# Autodesk Inventor assembly: Elevator Car with Plate
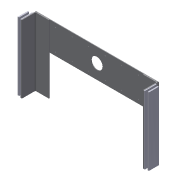
[picture p0: Inventor's stored thumbnail of the model, 180x180]
Saved by Autodesk Inventor 2015 (Build 190159000, 159)
## iProperties
Created: 2015-01-31
Part Number: Elevator Car with Plate
Document SubType Name: Assembly
Designer: Peter
Author: Peter
## Documents named in this file (3)
- T:\FILES\FIRST-Team-1719-CAD-Team\2015 Robot CAD\Lifter Super Structure\Elevator Car\Elevator Car with Plate.iam
- T:\FILES\FIRST-Team-1719-CAD-Team\2015 Robot CAD\Lifter Super Structure\Elevator Car\Elevator Car.iam
- T:\FILES\FIRST-Team-1719-CAD-Team\2015 Robot CAD\Lifter Super Structure\Elevator Cart\elevbackplt.ipt
## Components (3 placed, 2 different names)
1. Elevator Car:1 [sub-assembly] — Mate:1, Flush:3, Flush:4
2. Elevator Car:2 [sub-assembly] — Mate:2, Flush:1, Flush:2
3. elevbackplt:1 — Mate:1, Mate:2, Flush:1, Flush:2, Flush:3, Flush:4
## Relationships (6: Flush 4, Mate 2)
- Mate:1: Elevator Car:1 ↔ elevbackplt:1
- Mate:2: Elevator Car:2 ↔ elevbackplt:1
- Flush:1: Elevator Car:2 ↔ elevbackplt:1
- Flush:2: Elevator Car:2 ↔ elevbackplt:1
- Flush:3: Elevator Car:1 ↔ elevbackplt:1
- Flush:4: Elevator Car:1 ↔ elevbackplt:1
